# Autodesk Inventor assembly: 1102
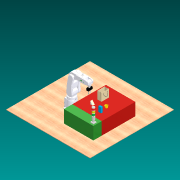
[picture p0: Inventor's stored thumbnail of the model, 180x180]
Saved by Autodesk Inventor 2022 (Build 260153000, 153)
## iProperties
Created: 2023-03-07
Part Number: 1102
Document SubType Name: Assembly
Designer: robot
Mass: 277297 g
Surface Area: 127951 cm^2
Volume: 277297 cm^3
Density: 1 g/cm^3
Author: robot
## Documents named in this file (25)
- C:\Users\ASUS\Desktop\312\1102.iam
- C:\Users\ASUS\Desktop\312\底板.ipt
- C:\Users\ASUS\Desktop\312\RA605-001.ipt
- C:\Users\ASUS\Desktop\312\RA605-002.ipt
- C:\Users\ASUS\Desktop\312\RA605-003.ipt
- C:\Users\ASUS\Desktop\312\RA605-004.ipt
- C:\Users\ASUS\Desktop\312\RA605-005.ipt
- C:\Users\ASUS\Desktop\312\RA605-006.ipt
- C:\Users\ASUS\Desktop\312\RA605-007.ipt
- C:\Users\ASUS\Desktop\312\桌1.ipt
- C:\Users\ASUS\Desktop\312\桌2.ipt
- C:\Users\ASUS\Desktop\312\杯子.ipt
- C:\Users\ASUS\Desktop\312\轉接版.ipt
- C:\Users\ASUS\Desktop\312\ARML.ipt
- C:\Users\ASUS\Desktop\312\ARMR.ipt
- C:\Users\ASUS\Desktop\312\汽缸.ipt
- C:\Users\ASUS\Desktop\312\杯蓋.ipt
- C:\Users\ASUS\Desktop\312\警示燈.ipt
- C:\Users\ASUS\Desktop\312\應變規.ipt
- C:\Users\ASUS\Desktop\312\夾爪2.ipt
- C:\Users\ASUS\Desktop\312\汽缸3.ipt
- C:\Users\ASUS\Desktop\312\袋子.ipt
- C:\Users\ASUS\Documents\零件2.ipt
- C:\Users\ASUS\Desktop\312\AI.ipt
- C:\Users\ASUS\Desktop\312\三明治.ipt
## Components (32 placed, 24 different names)
1. 底板:1 — 貼合:5, 貼合:6, 貼合:7, 貼合:44, 貼合:45
2. 桌1:1 — 貼合:4, 齊平:1, 齊平:2, 貼合:5, 貼合:7, 貼合:8, 貼合:9, 貼合:10, 貼合:11, 貼合:12, 貼合:39, 貼合:40, 貼合:41, 貼合:42, 貼合:43, 貼合:58, 貼合:59, 貼合:60, 貼合:61
3. 桌2:1 — 貼合:4, 齊平:1, 齊平:2, 貼合:6, 貼合:48
4. 杯子:1 — 貼合:8
5. 杯子:2 — 貼合:12
6. 杯子:3 — 貼合:11
7. 杯子:4 — 貼合:10
8. 杯子:5 — 貼合:9
9. 轉接版:1 — 貼合:24, 貼合:37, 貼合:46, 貼合:47, 貼合:55, 貼合:56, 貼合:57
10. ARML:1 — 貼合:36, 貼合:38, 角度:9
11. ARMR:1 — 貼合:35, 貼合:49, 貼合:50, 貼合:51, 角度:8
12. 汽缸:1 — 貼合:24, 貼合:35, 貼合:36, 貼合:37, 貼合:38, 角度:7, 貼合:50, 貼合:51, 角度:8, 角度:9
13. 杯蓋:1 — 貼合:39
14. 杯蓋:2 — 貼合:43
15. 杯蓋:3 — 貼合:42
16. 杯蓋:4 — 貼合:41
17. 杯蓋:5 — 貼合:40
18. RA605-001:1 — 貼合:44, 貼合:45
19. RA605-002:1
20. RA605-003:1
21. RA605-004:1
22. RA605-005:1 — 角度:7
23. RA605-006:1
24. RA605-007:1 — 貼合:46, 貼合:47
25. 警示燈:1 — 貼合:48
26. 應變規:1 — 貼合:49
27. 夾爪2:1 — 貼合:52, 貼合:53, 貼合:54
28. 汽缸3:1 — 貼合:52, 貼合:53, 貼合:54, 貼合:55, 貼合:56, 貼合:57
29. 袋子:1 — 貼合:58
30. 零件2:1 — 貼合:59
31. AI:1 — 貼合:60
32. 三明治:1 — 貼合:61
## Relationships (50: Mate 37, Insert 6, Angle 5, Flush 2)
- 貼合:4 [Mate]: 桌1:1 ↔ 桌2:1
- 齊平:1 [Flush]: 桌1:1 ↔ 桌2:1
- 齊平:2 [Flush]: 桌1:1 ↔ 桌2:1
- 貼合:5 [Mate]: 底板:1 ↔ 桌1:1
- 貼合:6 [Mate] (320 mm): 底板:1 ↔ 桌2:1
- 貼合:7 [Mate] (600 mm): 底板:1 ↔ 桌1:1
- 貼合:8 [Mate]: 桌1:1 ↔ 杯子:1
- 貼合:9 [Mate]: 桌1:1 ↔ 杯子:5
- 貼合:10 [Mate]: 桌1:1 ↔ 杯子:4
- 貼合:11 [Mate]: 桌1:1 ↔ 杯子:3
- 貼合:12 [Mate]: 桌1:1 ↔ 杯子:2
- 貼合:24 [Mate]: 轉接版:1 ↔ 汽缸:1
- 貼合:35 [Mate]: ARMR:1 ↔ 汽缸:1
- 貼合:36 [Mate]: ARML:1 ↔ 汽缸:1
- 貼合:37 [Mate]: 轉接版:1 ↔ 汽缸:1
- 貼合:38 [Mate]: ARML:1 ↔ 汽缸:1
- 貼合:39 [Mate] (90 mm): 桌1:1 ↔ 杯蓋:1
- 貼合:40 [Mate] (90 mm): 桌1:1 ↔ 杯蓋:5
- 貼合:41 [Mate] (90 mm): 桌1:1 ↔ 杯蓋:4
- 貼合:42 [Mate] (92 mm): 桌1:1 ↔ 杯蓋:3
- 貼合:43 [Mate] (90 mm): 桌1:1 ↔ 杯蓋:2
- [Insert]: RA605-004:1 ↔ RA605-005:1
- [Angle] (0 deg): RA605-001:1 ↔ RA605-005:1
- [Insert]: RA605-005:1 ↔ RA605-006:1
- [Insert]: RA605-006:1 ↔ RA605-007:1
- [Insert]: RA605-003:1 ↔ RA605-004:1
- [Insert]: RA605-002:1 ↔ RA605-003:1
- [Angle] (0 deg): RA605-005:1 ↔ RA605-006:1
- [Insert]: RA605-001:1 ↔ RA605-002:1
- 貼合:44 [Mate] (700 mm): 底板:1 ↔ RA605-001:1
- 貼合:45 [Mate]: 底板:1 ↔ RA605-001:1
- 貼合:46 [Mate]: 轉接版:1 ↔ RA605-007:1
- 貼合:47 [Mate]: 轉接版:1 ↔ RA605-007:1
- 角度:7 [Angle] (0 deg): 汽缸:1 ↔ RA605-005:1
- 貼合:48 [Mate]: 桌2:1 ↔ 警示燈:1
- 貼合:49 [Mate]: ARMR:1 ↔ 應變規:1
- 貼合:50 [Mate]: ARMR:1 ↔ 汽缸:1
- 貼合:51 [Mate]: ARMR:1 ↔ 汽缸:1
- 角度:8 [Angle] (-20 deg): ARMR:1 ↔ 汽缸:1
- 角度:9 [Angle] (20 deg): ARML:1 ↔ 汽缸:1
- 貼合:52 [Mate]: 夾爪2:1 ↔ 汽缸3:1
- 貼合:53 [Mate]: 夾爪2:1 ↔ 汽缸3:1
- 貼合:54 [Mate]: 夾爪2:1 ↔ 汽缸3:1
- 貼合:55 [Mate]: 轉接版:1 ↔ 汽缸3:1
- 貼合:56 [Mate]: 轉接版:1 ↔ 汽缸3:1
- 貼合:57 [Mate]: 轉接版:1 ↔ 汽缸3:1
- 貼合:58 [Mate]: 桌1:1 ↔ 袋子:1
- 貼合:59 [Mate]: 桌1:1 ↔ 零件2:1
- 貼合:60 [Mate]: 桌1:1 ↔ AI:1
- 貼合:61 [Mate]: 桌1:1 ↔ 三明治:1
